# Autodesk Inventor assembly: Full_HITscope_v0
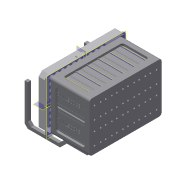
[picture p0: Inventor's stored thumbnail of the model, 180x180]
Saved by Autodesk Inventor 2019.4 (Build 234330000, 330)
## iProperties
Created: 2021-09-09
Part Number: Full_HITscope_v0
Material: Generisch
Document SubType Name: Assembly
Designer: Muriel
Mass: 256.869 g
Surface Area: 2541.25 cm^2
Volume: 256.869 cm^3
Density: 1 g/cm^3
Author: Muriel
## Documents named in this file (7)
- C:\Users\diederichbenedict\Dropbox\Dokumente\Promotion\PROJECTS\Omniscope\INVENTOR\Full_HITscope_v0.iam
- C:\Users\diederichbenedict\Dropbox\Dokumente\Promotion\PROJECTS\Omniscope\INVENTOR\Assembly_Omniscope_v1.iam
- C:\Users\diederichbenedict\Dropbox\Dokumente\Promotion\PROJECTS\Omniscope\INVENTOR\05_Omniscope_base_v1.ipt
- C:\Users\diederichbenedict\Dropbox\Dokumente\Promotion\PROJECTS\Omniscope\INVENTOR\06_Omniscope_lid_lenses.ipt
- C:\Users\diederichbenedict\Dropbox\Dokumente\Promotion\PROJECTS\Omniscope\INVENTOR\00_OV_lens.ipt
- C:\Users\diederichbenedict\Dropbox\Dokumente\Promotion\PROJECTS\Omniscope\INVENTOR\00_MTP_96-welplate.ipt
- C:\Users\diederichbenedict\Dropbox\Dokumente\Promotion\PROJECTS\Omniscope\INVENTOR\07_Omnivision_Lamp_arm.ipt
## Components (18 placed, 6 different names)
1. 05_Omniscope_base_v1:1 — Fluchtend:1, Fluchtend:2, Fluchtend:3, Fluchtend:4, Winkel:1, Fluchtend:5, Fluchtend:6, Einfügen:2
2. 06_Omniscope_lid_lenses:1 — Fluchtend:3, Fluchtend:4, Einfügen:1, Passend:1, Passend:2, Passend:3
3. 00_OV_lens:1 — Einfügen:1
4. 00_MTP_96-welplate:1 — Passend:1, Winkel:1, Passend:2, Passend:3
5. 07_Omnivision_Lamp_arm:1 — Fluchtend:5, Fluchtend:6
6. 07_Omnivision_Lamp_arm:2 — Einfügen:2, Winkel:2
7. Assembly_Omniscope_v1:1 [sub-assembly]
8. Assembly_Omniscope_v1:2 [sub-assembly]
9. Assembly_Omniscope_v1:3 [sub-assembly]
10. Assembly_Omniscope_v1:4 [sub-assembly]
11. Assembly_Omniscope_v1:5 [sub-assembly]
12. Assembly_Omniscope_v1:6 [sub-assembly]
13. Assembly_Omniscope_v1:7 [sub-assembly]
14. Assembly_Omniscope_v1:8 [sub-assembly]
15. Assembly_Omniscope_v1:9 [sub-assembly]
16. Assembly_Omniscope_v1:10 [sub-assembly]
17. Assembly_Omniscope_v1:11 [sub-assembly] — Fluchtend:1, Fluchtend:2
18. Assembly_Omniscope_v1:12 [sub-assembly] — Winkel:2
## Component patterns: (12 elements, first: Assembly_Omniscope_v1:1)
## Relationships (13: Flush 6, Mate 3, Insert 2, Angle 2)
- Fluchtend:1 [Flush]: 05_Omniscope_base_v1:1 ↔ Assembly_Omniscope_v1:11
- Fluchtend:2 [Flush]: 05_Omniscope_base_v1:1 ↔ Assembly_Omniscope_v1:11
- Fluchtend:3 [Flush]: 05_Omniscope_base_v1:1 ↔ 06_Omniscope_lid_lenses:1
- Fluchtend:4 [Flush]: 05_Omniscope_base_v1:1 ↔ 06_Omniscope_lid_lenses:1
- Einfügen:1 [Insert]: 06_Omniscope_lid_lenses:1 ↔ 00_OV_lens:1
- Passend:1 [Mate]: 06_Omniscope_lid_lenses:1 ↔ 00_MTP_96-welplate:1
- Winkel:1 [Angle] (0 deg): 05_Omniscope_base_v1:1 ↔ 00_MTP_96-welplate:1
- Passend:2 [Mate]: 06_Omniscope_lid_lenses:1 ↔ 00_MTP_96-welplate:1
- Passend:3 [Mate]: 06_Omniscope_lid_lenses:1 ↔ 00_MTP_96-welplate:1
- Fluchtend:5 [Flush]: 05_Omniscope_base_v1:1 ↔ 07_Omnivision_Lamp_arm:1
- Fluchtend:6 [Flush]: 05_Omniscope_base_v1:1 ↔ 07_Omnivision_Lamp_arm:1
- Einfügen:2 [Insert]: 05_Omniscope_base_v1:1 ↔ 07_Omnivision_Lamp_arm:2
- Winkel:2 [Angle] (0 deg): 07_Omnivision_Lamp_arm:2 ↔ Assembly_Omniscope_v1:12
